# Autodesk Inventor assembly: Assembly1
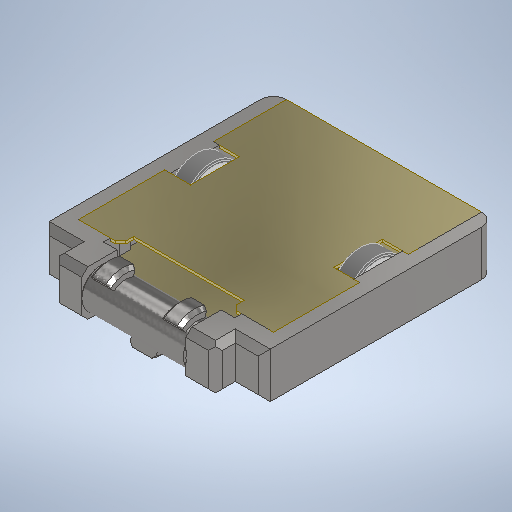
[picture p0: Inventor's stored thumbnail of the model, 512x512]
Saved by Autodesk Inventor 2025 (Build 290162000, 162)
## iProperties
Created: 2026-06-07
Part Number: Assembly1
Document SubType Name: Assembly
Designer: user
Author: user
## Documents named in this file (8)
- C:\Users\user\Documents\Gabriel\Proyectos\Robot de pelea\Assembly1.iam
- C:\Users\user\Documents\Gabriel\Proyectos\Robot de pelea\Part2.ipt
- C:\Users\user\Documents\Gabriel\Proyectos\Robot de pelea\Part1.ipt
- C:\Users\user\Documents\Gabriel\Proyectos\Robot de pelea\Part6.ipt
- C:\Users\user\Documents\Gabriel\Proyectos\Robot de pelea\Part5.ipt
- C:\Users\user\Documents\Gabriel\Proyectos\Robot de pelea\Part4.ipt
- C:\Users\user\Documents\Gabriel\Proyectos\Robot de pelea\Part3.ipt
- C:\Users\user\Documents\Gabriel\Proyectos\Robot de pelea\Assembly1\Design Accelerator\Bearing2.iam
## Components (13 placed, 7 different names)
1. Part2:1 — Mate:1, Mate:2, Mate:3, Mate:4, Mate:9, Mate:15, Mate:21, Mate:22, Mate:25, Flush:5
2. Part2:2 — Mate:5, Mate:6, Mate:7, Mate:11, Mate:13, Mate:20, Mate:23, Mate:24, Mate:26
3. Part1:1 — Mate:1, Mate:2, Mate:3, Flush:1, Flush:2, Mate:5, Mate:6, Mate:7
4. Part1:2 — Flush:1, Mate:4, Flush:2, Mate:8, Mate:10, Flush:4
5. Part6:1 — Mate:11, Flush:3, Flush:4, Mate:12
6. Part6:2 — Mate:8, Mate:9, Mate:10, Flush:3, Mate:14
7. Part5:1 — Mate:12, Mate:13, Mate:16, Mate:19
8. Part5:2 — Mate:14, Mate:15, Mate:17, Mate:18
9. Part4:1 — Mate:17, Mate:18, Mate:21
10. Part4:2 — Mate:16, Mate:19, Mate:20
11. Part3:1 — Mate:22, Mate:26
12. Bearing:1 [sub-assembly] — Mate:23, Mate:24
13. Bearing:2 [sub-assembly] — Mate:25, Flush:5
## Relationships (31: Mate 26, Flush 5)
- Mate:1: Part2:1 ↔ Part1:1
- Mate:2: Part2:1 ↔ Part1:1
- Mate:3: Part2:1 ↔ Part1:1
- Flush:1: Part1:1 ↔ Part1:2
- Mate:4: Part2:1 ↔ Part1:2
- Flush:2: Part1:1 ↔ Part1:2
- Mate:5: Part2:2 ↔ Part1:1
- Mate:6: Part2:2 ↔ Part1:1
- Mate:7: Part2:2 ↔ Part1:1
- Mate:8 (1 mm): Part1:2 ↔ Part6:2
- Mate:9 (35 mm): Part2:1 ↔ Part6:2
- Mate:10 (7.25 mm): Part1:2 ↔ Part6:2
- Mate:11 (35 mm): Part2:2 ↔ Part6:1
- Flush:3: Part6:1 ↔ Part6:2
- Flush:4 (-5 mm): Part1:2 ↔ Part6:1
- Mate:12: Part6:1 ↔ Part5:1
- Mate:13 (2 mm): Part2:2 ↔ Part5:1
- Mate:14: Part6:2 ↔ Part5:2
- Mate:15 (2 mm): Part2:1 ↔ Part5:2
- Mate:16: Part5:1 ↔ Part4:2
- Mate:17: Part5:2 ↔ Part4:1
- Mate:18: Part5:2 ↔ Part4:1
- Mate:19: Part5:1 ↔ Part4:2
- Mate:20 (1 mm): Part2:2 ↔ Part4:2
- Mate:21 (1 mm): Part2:1 ↔ Part4:1
- Mate:22: Part2:1 ↔ Part3:1
- Mate:23: Part2:2 ↔ Bearing:1
- Mate:24: Part2:2 ↔ Bearing:1
- Mate:25: Part2:1 ↔ Bearing:2
- Flush:5: Part2:1 ↔ Bearing:2
- Mate:26: Part2:2 ↔ Part3:1
